# Autodesk Inventor assembly: hopper_with_connector
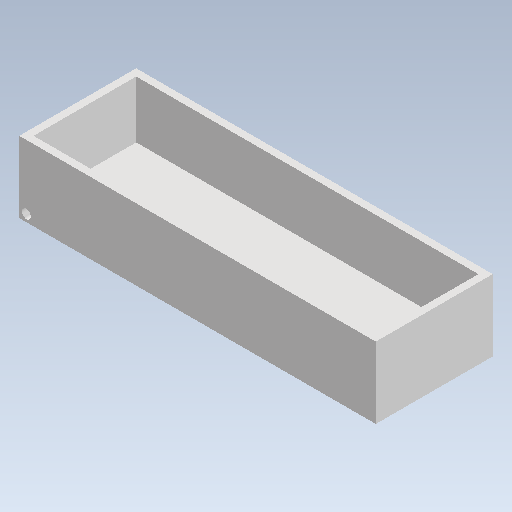
[picture p0: Inventor's stored thumbnail of the model, 512x512]
Saved by Autodesk Inventor 2021 (Build 250183000, 183)
## iProperties
Created: 2021-02-07
Part Number: hopper_with_connector
Document SubType Name: Assembly
Designer: chris
Mass: 335.798 g
Surface Area: 1032.8 cm^2
Volume: 335.798 cm^3
Density: 1 g/cm^3
Author: chris
## Documents named in this file (3)
- C:\Users\chris\Desktop\Project 3 Device\hopper_with_connector.iam
- C:\Users\chris\Desktop\Project 3 Device\GivenHopper (to be modified by your team).ipt
- C:\Users\chris\Desktop\Project 3 Device\Connector.ipt
## Components (3 placed, 2 different names)
1. GivenHopper (to be modified by your team):1 — Mate:1, Mate:2, Flush:1, Flush:3
2. Connector:1 — Mate:2, Flush:2, Mate:3
3. Connector:2 — Mate:1, Flush:1, Flush:2, Mate:3, Flush:3
## Relationships (6: Mate 3, Flush 3)
- Mate:1: GivenHopper (to be modified by your team):1 ↔ Connector:2
- Mate:2: GivenHopper (to be modified by your team):1 ↔ Connector:1
- Flush:1 (116 mm): GivenHopper (to be modified by your team):1 ↔ Connector:2
- Flush:2: Connector:1 ↔ Connector:2
- Mate:3 (10 mm): Connector:1 ↔ Connector:2
- Flush:3 (21 mm): GivenHopper (to be modified by your team):1 ↔ Connector:2
